# Autodesk Inventor assembly: Assembly
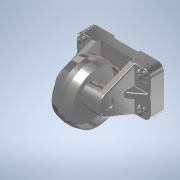
[picture p0: Inventor's stored thumbnail of the model, 180x180]
Saved by Autodesk Inventor 2020 (Build 240168000, 168)
## iProperties
Created: 2021-06-13
Part Number: Assembly
Document SubType Name: Assembly
Designer: joelm
Author: joelm
## Documents named in this file (5)
- D:\Carreer 4.1\Manufacturing Tech\DieSetProject-20210729T070551Z-001\DieSetProject\DieSet\Assembly.iam
- D:\Carreer 4.1\Manufacturing Tech\DieSetProject-20210729T070551Z-001\DieSetProject\DieSet\axle.ipt
- D:\Carreer 4.1\Manufacturing Tech\DieSetProject-20210729T070551Z-001\DieSetProject\DieSet\axleSupport.ipt
- D:\Carreer 4.1\Manufacturing Tech\DieSetProject-20210729T070551Z-001\DieSetProject\DieSet\topPlate.ipt
- D:\Carreer 4.1\Manufacturing Tech\DieSetProject-20210729T070551Z-001\DieSetProject\DieSet\wheel.ipt
## Components (5 placed, 4 different names)
1. axle:1 — Mate:1, Mate:2, Flush:1
2. axleSupport:1 — Mate:2, Flush:1, Mate:4, Mate:6, Mate:7, Flush:2
3. topPlate:1 — Mate:5, Mate:6, Mate:7, Flush:2, Flush:3
4. wheel:1 — Mate:1, Mate:3, Mate:4
5. axleSupport:2 — Mate:3, Mate:5, Flush:3
## Relationships (10: Mate 7, Flush 3)
- Mate:1: axle:1 ↔ wheel:1
- Mate:2: axle:1 ↔ axleSupport:1
- Mate:3: wheel:1 ↔ axleSupport:2
- Flush:1 (-2 mm): axle:1 ↔ axleSupport:1
- Mate:4: axleSupport:1 ↔ wheel:1
- Mate:5: topPlate:1 ↔ axleSupport:2
- Mate:6: axleSupport:1 ↔ topPlate:1
- Mate:7: axleSupport:1 ↔ topPlate:1
- Flush:2: axleSupport:1 ↔ topPlate:1
- Flush:3: topPlate:1 ↔ axleSupport:2
